# Autodesk Inventor assembly: Portalfraese_V2_Z-Axis
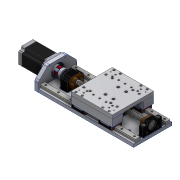
[picture p0: Inventor's stored thumbnail of the model, 180x180]
Saved by Autodesk Inventor 2016 (Build 200138000, 138)
## iProperties
Created: 2015-07-20
Part Number: Portalfraese_V2_Z-Axis
Document SubType Name: Assembly
Mass: 4544.64 g
Surface Area: 3288.98 cm^2
Volume: 1436.27 cm^3
Density: 3.16419 g/cm^3
## Documents named in this file (11)
- E:\GitHub\CNC-Router_Z-Axis\Portalfraese_V2_Z-Axis.iam
- E:\GitHub\CNC-Router_Z-Axis\Linearfuehrung Bosch Rexroth R0442.iam
- E:\GitHub\CNC-Router_Z-Axis\ISSOKU_Ballscrew_D12x160_05_590104-13.iam
- E:\GitHub\CNC-Router_Z-Axis\Grundplatte.ipt
- E:\GitHub\Buy-Parts\Stepper_Nema23_23HS33-4008S.ipt
- E:\GitHub\CNC-Router_Z-Axis\Motorhalterung.ipt
- E:\GitHub\Buy-Parts\Klauenkupplung_d6-35_d8.ipt
- E:\GitHub\CNC-Router_Z-Axis\Schlitten.iam
- C:\Dropbox\Inventor\Projects\Fraese_konventionell\Spindelhalter.iam
- C:\Dropbox\Inventor\Projects\Portalfraese_V2\Zwischenplatte.ipt
- C:\Dropbox\Inventor\Projects\001_EK-Teile\Kress 1050 FME.ipt
## Components (11 placed, 10 different names)
1. ISSOKU_Ballscrew_D12x160_05_590104-13:1 [sub-assembly] — Mate:3, Mate:5, Mate:8, Insert:1, Mate:16, Mate:17, Flush:12, Mate:22
2. Linearfuehrung Bosch Rexroth R0442:1 [sub-assembly] — Mate:4, Flush:8, Mate:21, Mate:23, Mate:27
3. Linearfuehrung Bosch Rexroth R0442:2 [sub-assembly] — Mate:24, Mate:26, Mate:28, Mate:29, Mate:30
4. Grundplatte:1 — Mate:3, Mate:4, Flush:8, Mate:5, Angle:1, Mate:10, Flush:10, Mate:16, Mate:23, Mate:24, Mate:28
5. Stepper_Nema23_23HS33-4008S:1 — Mate:8, Angle:1, Mate:11, Mate:14
6. Motorhalterung:1 — Mate:10, Mate:11, Flush:10, Mate:14, Mate:26
7. Klauenkupplung_d6-35_d8:1 — Insert:1
8. Schlitten:1 [sub-assembly] — Mate:17, Flush:12, Mate:20, Mate:21, Mate:22, Mate:27, Mate:29, Mate:30, Mate:31, Mate:32
9. Spindelhalter:1 [sub-assembly] — Insert:2, Mate:19, Insert:3
10. Zwischenplatte:1 — Insert:2, Mate:19, Mate:20, Mate:31, Mate:32
11. Kress 1050 FME:1 — Insert:3
## Relationships (29: Mate 22, Flush 3, Insert 3, Angle 1)
- Mate:3: ISSOKU_Ballscrew_D12x160_05_590104-13:1 ↔ Grundplatte:1
- Mate:4: Linearfuehrung Bosch Rexroth R0442:1 ↔ Grundplatte:1
- Flush:8: Linearfuehrung Bosch Rexroth R0442:1 ↔ Grundplatte:1
- Mate:5 (3 mm): ISSOKU_Ballscrew_D12x160_05_590104-13:1 ↔ Grundplatte:1
- Mate:8: ISSOKU_Ballscrew_D12x160_05_590104-13:1 ↔ Stepper_Nema23_23HS33-4008S:1
- Angle:1 (0 deg): Grundplatte:1 ↔ Stepper_Nema23_23HS33-4008S:1
- Mate:10: Grundplatte:1 ↔ Motorhalterung:1
- Mate:11: Stepper_Nema23_23HS33-4008S:1 ↔ Motorhalterung:1
- Flush:10: Grundplatte:1 ↔ Motorhalterung:1
- Insert:1 (1.5 mm): ISSOKU_Ballscrew_D12x160_05_590104-13:1 ↔ Klauenkupplung_d6-35_d8:1
- Mate:14: Stepper_Nema23_23HS33-4008S:1 ↔ Motorhalterung:1
- Mate:16: ISSOKU_Ballscrew_D12x160_05_590104-13:1 ↔ Grundplatte:1
- Mate:17: ISSOKU_Ballscrew_D12x160_05_590104-13:1 ↔ Schlitten:1
- Flush:12: ISSOKU_Ballscrew_D12x160_05_590104-13:1 ↔ Schlitten:1
- Insert:2: Spindelhalter:1 ↔ Zwischenplatte:1
- Mate:19: Spindelhalter:1 ↔ Zwischenplatte:1
- Mate:20: Schlitten:1 ↔ Zwischenplatte:1
- Insert:3: Spindelhalter:1 ↔ Kress 1050 FME:1
- Mate:21: Linearfuehrung Bosch Rexroth R0442:1 ↔ Schlitten:1
- Mate:22: ISSOKU_Ballscrew_D12x160_05_590104-13:1 ↔ Schlitten:1
- Mate:23: Linearfuehrung Bosch Rexroth R0442:1 ↔ Grundplatte:1
- Mate:24: Linearfuehrung Bosch Rexroth R0442:2 ↔ Grundplatte:1
- Mate:26: Linearfuehrung Bosch Rexroth R0442:2 ↔ Motorhalterung:1
- Mate:27: Linearfuehrung Bosch Rexroth R0442:1 ↔ Schlitten:1
- Mate:28: Linearfuehrung Bosch Rexroth R0442:2 ↔ Grundplatte:1
- Mate:29: Linearfuehrung Bosch Rexroth R0442:2 ↔ Schlitten:1
- Mate:30: Linearfuehrung Bosch Rexroth R0442:2 ↔ Schlitten:1
- Mate:31: Schlitten:1 ↔ Zwischenplatte:1
- Mate:32: Schlitten:1 ↔ Zwischenplatte:1
